# Autodesk Inventor assembly: Top Conveyor Roller Wheel Assembly
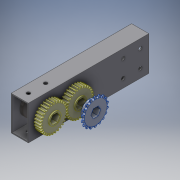
[picture p0: Inventor's stored thumbnail of the model, 180x180]
Saved by Autodesk Inventor 2018 (Build 220112000, 112)
## iProperties
Created: 2020-02-21
Part Number: Top Conveyor Roller Wheel Assembly
Document SubType Name: Assembly
Designer: T3500STATIC
Author: T3500STATIC
## Documents named in this file (5)
- C:\Users\T3500STATIC\Documents\GitHub\2020CAD\Gabriel Inventor Files (Shooter, Drivebase)\Shooter Curve Assembly\Part Files\Top Conveyor Roller Wheel Assembly.iam
- C:\Users\T3500STATIC\Documents\GitHub\2020CAD\Gabriel Inventor Files (Shooter, Drivebase)\Shooter Curve Assembly\Part Files\Top Roller Wheel Mount.ipt
- C:\Users\T3500STATIC\Documents\GitHub\2020CAD\Gabriel Inventor Files (Shooter, Drivebase)\Shooter Curve Assembly\Part Files\30t_Steel_Spur_Gear_20_DP_1_2_Hex_Bore_217-5469.ipt
- C:\Users\T3500STATIC\Documents\GitHub\2020CAD\Gabriel Inventor Files (Shooter, Drivebase)\Shooter Curve Assembly\Part Files\_18t_Aluminum_Hub_Sprocket_25_Chain_1_2_Hex_Bore_217-3488.ipt
- C:\Users\T3500STATIC\Documents\GitHub\2020CAD\Gabriel Inventor Files (Shooter, Drivebase)\Drivebase Assembly\Part Files\FR8ZZ Hex Bearing.ipt
## Components (8 placed, 4 different names)
1. Top Roller Wheel Mount:1 — Mate:1, Mate:2, Mate:3, Mate:4, Mate:8, Mate:9
2. 30t_Steel_Spur_Gear_20_DP_1_2_Hex_Bore_217-5469:1 — Flush:1, Flush:2, Mate:5, Mate:7, Flush:5, Flush:6
3. 30t_Steel_Spur_Gear_20_DP_1_2_Hex_Bore_217-5469:2 — Mate:6, Flush:3, Flush:4
4. _18t_Aluminum_Hub_Sprocket_25_Chain_1_2_Hex_Bore_217-3488:1 — Mate:7, Flush:5, Flush:6
5. FR8ZZ Hex Bearing:1 — Mate:2, Mate:6, Flush:3, Flush:4, Mate:9
6. FR8ZZ Hex Bearing:2 — Mate:1, Flush:1, Flush:2, Mate:5, Mate:8
7. FR8ZZ Hex Bearing:3 — Mate:4
8. FR8ZZ Hex Bearing:4 — Mate:3
## Relationships (15: Mate 9, Flush 6)
- Mate:1: Top Roller Wheel Mount:1 ↔ FR8ZZ Hex Bearing:2
- Mate:2: Top Roller Wheel Mount:1 ↔ FR8ZZ Hex Bearing:1
- Mate:3: Top Roller Wheel Mount:1 ↔ FR8ZZ Hex Bearing:4
- Mate:4: Top Roller Wheel Mount:1 ↔ FR8ZZ Hex Bearing:3
- Flush:1: 30t_Steel_Spur_Gear_20_DP_1_2_Hex_Bore_217-5469:1 ↔ FR8ZZ Hex Bearing:2
- Flush:2: 30t_Steel_Spur_Gear_20_DP_1_2_Hex_Bore_217-5469:1 ↔ FR8ZZ Hex Bearing:2
- Mate:5: 30t_Steel_Spur_Gear_20_DP_1_2_Hex_Bore_217-5469:1 ↔ FR8ZZ Hex Bearing:2
- Mate:6: 30t_Steel_Spur_Gear_20_DP_1_2_Hex_Bore_217-5469:2 ↔ FR8ZZ Hex Bearing:1
- Flush:3: 30t_Steel_Spur_Gear_20_DP_1_2_Hex_Bore_217-5469:2 ↔ FR8ZZ Hex Bearing:1
- Flush:4: 30t_Steel_Spur_Gear_20_DP_1_2_Hex_Bore_217-5469:2 ↔ FR8ZZ Hex Bearing:1
- Mate:7 (12.7 mm): 30t_Steel_Spur_Gear_20_DP_1_2_Hex_Bore_217-5469:1 ↔ _18t_Aluminum_Hub_Sprocket_25_Chain_1_2_Hex_Bore_217-3488:1
- Flush:5: 30t_Steel_Spur_Gear_20_DP_1_2_Hex_Bore_217-5469:1 ↔ _18t_Aluminum_Hub_Sprocket_25_Chain_1_2_Hex_Bore_217-3488:1
- Flush:6: 30t_Steel_Spur_Gear_20_DP_1_2_Hex_Bore_217-5469:1 ↔ _18t_Aluminum_Hub_Sprocket_25_Chain_1_2_Hex_Bore_217-3488:1
- Mate:8: Top Roller Wheel Mount:1 ↔ FR8ZZ Hex Bearing:2
- Mate:9: Top Roller Wheel Mount:1 ↔ FR8ZZ Hex Bearing:1
